# Autodesk Inventor assembly: ASM1001-210 1U Board
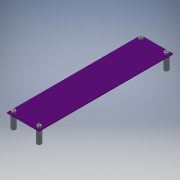
[picture p0: Inventor's stored thumbnail of the model, 180x180]
Saved by Autodesk Inventor 2019 (Build 230136000, 136)
## iProperties
Created: 2019-07-02
Part Number: ASM1001-210 1U Board
Document SubType Name: Assembly
Designer: james
Author: james
## Documents named in this file (4)
- F:\JimsDesign\P1001-16bit-CPU\ASM1001-210 1U Board.iam
- F:\JimsDesign\P1001-16bit-CPU\PRT1001-210 1U Board.ipt
- F:\JimsDesign\P1001-16bit-CPU\92080A713_ZNC-PLTD BRASS FEM THRDED HEX STANDOFF.ipt
- F:\JimsDesign\P1001-16bit-CPU\90349A103_METRIC BRASS SOCKET HEAD SCREW.ipt
## Components (9 placed, 3 different names)
1. PRT1001-210 1U Board:1 — Mate:1, Mate:2, Mate:3, Mate:4, Mate:5, Mate:6, Mate:7, Mate:8, Mate:9, Mate:10, Mate:11, Mate:12, Mate:13, Mate:14, Mate:15, Mate:16
2. 92080A713_ZNC-PLTD BRASS FEM THRDED HEX STANDOFF:1 — Mate:4, Mate:8
3. 92080A713_ZNC-PLTD BRASS FEM THRDED HEX STANDOFF:2 — Mate:3, Mate:7
4. 92080A713_ZNC-PLTD BRASS FEM THRDED HEX STANDOFF:3 — Mate:2, Mate:6
5. 92080A713_ZNC-PLTD BRASS FEM THRDED HEX STANDOFF:4 — Mate:1, Mate:5
6. 90349A103_METRIC BRASS SOCKET HEAD SCREW:1 — Mate:9, Mate:14
7. 90349A103_METRIC BRASS SOCKET HEAD SCREW:2 — Mate:10, Mate:13
8. 90349A103_METRIC BRASS SOCKET HEAD SCREW:3 — Mate:11, Mate:15
9. 90349A103_METRIC BRASS SOCKET HEAD SCREW:4 — Mate:12, Mate:16
## Relationships (16: Mate 16)
- Mate:1: PRT1001-210 1U Board:1 ↔ 92080A713_ZNC-PLTD BRASS FEM THRDED HEX STANDOFF:4
- Mate:2: PRT1001-210 1U Board:1 ↔ 92080A713_ZNC-PLTD BRASS FEM THRDED HEX STANDOFF:3
- Mate:3: PRT1001-210 1U Board:1 ↔ 92080A713_ZNC-PLTD BRASS FEM THRDED HEX STANDOFF:2
- Mate:4: PRT1001-210 1U Board:1 ↔ 92080A713_ZNC-PLTD BRASS FEM THRDED HEX STANDOFF:1
- Mate:5: PRT1001-210 1U Board:1 ↔ 92080A713_ZNC-PLTD BRASS FEM THRDED HEX STANDOFF:4
- Mate:6: PRT1001-210 1U Board:1 ↔ 92080A713_ZNC-PLTD BRASS FEM THRDED HEX STANDOFF:3
- Mate:7: PRT1001-210 1U Board:1 ↔ 92080A713_ZNC-PLTD BRASS FEM THRDED HEX STANDOFF:2
- Mate:8: PRT1001-210 1U Board:1 ↔ 92080A713_ZNC-PLTD BRASS FEM THRDED HEX STANDOFF:1
- Mate:9: PRT1001-210 1U Board:1 ↔ 90349A103_METRIC BRASS SOCKET HEAD SCREW:1
- Mate:10: PRT1001-210 1U Board:1 ↔ 90349A103_METRIC BRASS SOCKET HEAD SCREW:2
- Mate:11: PRT1001-210 1U Board:1 ↔ 90349A103_METRIC BRASS SOCKET HEAD SCREW:3
- Mate:12: PRT1001-210 1U Board:1 ↔ 90349A103_METRIC BRASS SOCKET HEAD SCREW:4
- Mate:13: PRT1001-210 1U Board:1 ↔ 90349A103_METRIC BRASS SOCKET HEAD SCREW:2
- Mate:14: PRT1001-210 1U Board:1 ↔ 90349A103_METRIC BRASS SOCKET HEAD SCREW:1
- Mate:15: PRT1001-210 1U Board:1 ↔ 90349A103_METRIC BRASS SOCKET HEAD SCREW:3
- Mate:16: PRT1001-210 1U Board:1 ↔ 90349A103_METRIC BRASS SOCKET HEAD SCREW:4
